# Autodesk Inventor assembly: motor_test
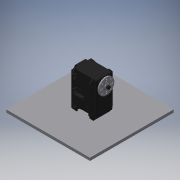
[picture p0: Inventor's stored thumbnail of the model, 180x180]
Saved by Autodesk Inventor 2018 (Build 220112000, 112)
## iProperties
Created: 2020-02-21
Part Number: motor_test
Document SubType Name: Assembly
Designer: bitbots
Author: bitbots
## Documents named in this file (3)
- C:\Users\bitbots\Desktop\bitbots_hardware\motor_tester\motor_test.iam
- C:\Users\bitbots\Desktop\bitbots_hardware\wolfgang\assembly\motors\MX106\MX-106_with_horn.iam
- C:\Users\bitbots\Desktop\bitbots_hardware\motor_tester\base.ipt
## Components (2 placed, 2 different names)
1. MX-106_with_horn:1 [sub-assembly] — Flush:4, Mate:1, Mate:2
2. base:1 — Flush:1, Flush:2, Flush:3, Flush:4, Mate:1
## Relationships (6: Flush 4, Mate 2)
- Flush:1: base:1
- Flush:2: base:1
- Flush:3: base:1
- Flush:4: MX-106_with_horn:1 ↔ base:1
- Mate:1: MX-106_with_horn:1 ↔ base:1
- Mate:2: MX-106_with_horn:1
